# Autodesk Inventor assembly: Assembly1
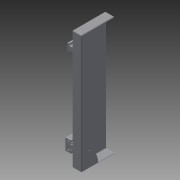
[picture p0: Inventor's stored thumbnail of the model, 180x180]
Saved by Autodesk Inventor 2015 SP1 (Build 190203100, 203)
## iProperties
Created: 2015-12-22
Part Number: Assembly1
Document SubType Name: Assembly
Designer: pc
Author: pc
## Documents named in this file (3)
- C:\Users\pc\Desktop\piezas\coche\Assembly1.iam
- C:\Users\pc\Desktop\piezas\coche\movil.ipt
- C:\Users\pc\Desktop\piezas\coche\guia.ipt
## Components (2 placed, 2 different names)
1. movil:1 — Mate:2, Flush:1
2. guia:1 — Mate:2, Flush:1
## Relationships (2: Mate 1, Flush 1)
- Mate:2: movil:1 ↔ guia:1
- Flush:1: movil:1 ↔ guia:1
